# Autodesk Inventor assembly: Puszka
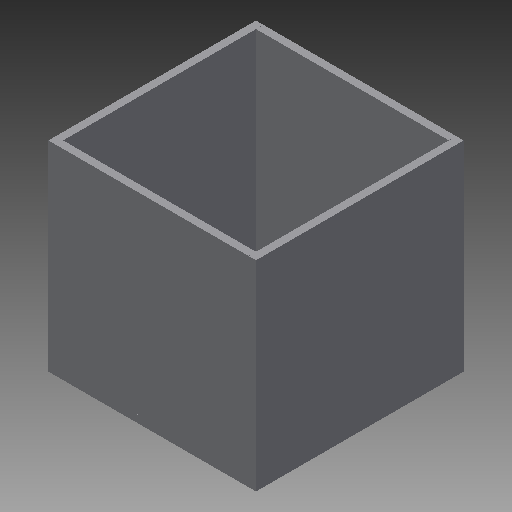
[picture p0: Inventor's stored thumbnail of the model, 512x512]
Saved by Autodesk Inventor 2018 (Build 220112000, 112)
## iProperties
Created: 2018-10-22
Part Number: Puszka
Material: Ogólny
Document SubType Name: Assembly
Designer: EWA
Author: EWA
## Documents named in this file (4)
- C:\Users\EWA\Documents\Inventor\Kostka\Puszka.iam
- C:\Users\EWA\Documents\Inventor\Kostka\Sciana_156x156.ipt
- C:\Users\EWA\Documents\Inventor\Kostka\Sciana_168x156.ipt
- C:\Users\EWA\Documents\Inventor\Kostka\Sciana_168x168.ipt
## Components (5 placed, 3 different names)
1. Sciana_156x156:1 — Zestawiający:3, Zestawiający:4, Równoległy:5
2. Sciana_168x156:1 — Zestawiający:2, Równoległy:3, Równoległy:4
3. Sciana_168x168:1 — Zestawiający:1, Równoległy:1, Równoległy:2, Zestawiający:2, Równoległy:3, Równoległy:4, Zestawiający:3, Równoległy:5, Równoległy:6, Zestawiający:5
4. Sciana_156x156:2 — Równoległy:6, Zestawiający:5, Zestawiający:6
5. Sciana_168x156:2 — Zestawiający:1, Równoległy:1, Równoległy:2, Zestawiający:4, Zestawiający:6
## Relationships (12: Mate 6, Flush 6)
- Zestawiający:1 [Mate]: Sciana_168x168:1 ↔ Sciana_168x156:2
- Równoległy:1 [Flush]: Sciana_168x168:1 ↔ Sciana_168x156:2
- Równoległy:2 [Flush]: Sciana_168x168:1 ↔ Sciana_168x156:2
- Zestawiający:2 [Mate]: Sciana_168x156:1 ↔ Sciana_168x168:1
- Równoległy:3 [Flush]: Sciana_168x156:1 ↔ Sciana_168x168:1
- Równoległy:4 [Flush]: Sciana_168x156:1 ↔ Sciana_168x168:1
- Zestawiający:3 [Mate]: Sciana_156x156:1 ↔ Sciana_168x168:1
- Zestawiający:4 [Mate]: Sciana_156x156:1 ↔ Sciana_168x156:2
- Równoległy:5 [Flush]: Sciana_156x156:1 ↔ Sciana_168x168:1
- Równoległy:6 [Flush]: Sciana_168x168:1 ↔ Sciana_156x156:2
- Zestawiający:5 [Mate]: Sciana_168x168:1 ↔ Sciana_156x156:2
- Zestawiający:6 [Mate]: Sciana_156x156:2 ↔ Sciana_168x156:2
